# Autodesk Inventor assembly: Assembly
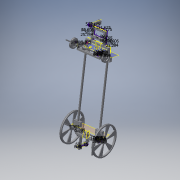
[picture p0: Inventor's stored thumbnail of the model, 180x180]
Saved by Autodesk Inventor 2018 (Build 220112000, 112)
## iProperties
Created: 2017-11-06
Part Number: Assembly
Document SubType Name: Assembly
Designer: David Cutting
Author: David Cutting
## Documents named in this file (19)
- C:\Users\Prakash\Documents\Inventor\MousetrapGit\Assembly.iam
- C:\Users\Prakash\Documents\Inventor\MousetrapGit\frontChassis_final.ipt
- C:\Users\Prakash\Documents\Inventor\MousetrapGit\carbonFiberTube.ipt
- C:\Users\Prakash\Documents\Inventor\MousetrapGit\clampCap.ipt
- C:\Users\Prakash\Documents\Inventor\MousetrapGit\rearChassis_final.ipt
- C:\Users\Prakash\Documents\Inventor\MousetrapGit\535018\bearings.ipt
- C:\Users\Prakash\Documents\Inventor\MousetrapGit\98873A200_MOISTURE-RESISTANT ACETAL THREADED ROD.ipt
- C:\Users\Prakash\Documents\Inventor\MousetrapGit\nutSecurer.ipt
- C:\Users\Prakash\Documents\Inventor\MousetrapGit\99223A029_ACETAL HEX NUT.ipt
- C:\Users\Prakash\Documents\Inventor\MousetrapGit\wheel.ipt
- C:\Users\Prakash\Documents\Inventor\MousetrapGit\spindleRod.ipt
- C:\Users\Prakash\Documents\Inventor\MousetrapGit\wheelSpindle.ipt
- C:\Users\Prakash\Documents\Inventor\MousetrapGit\intermediateSpindle.ipt
- C:\Users\Prakash\Documents\Inventor\MousetrapGit\wingnut_final.ipt
- C:\Users\Prakash\Documents\Inventor\MousetrapGit\washeript.ipt
- C:\Users\Prakash\Documents\Inventor\MousetrapGit\smallWheel.ipt
- C:\Users\Prakash\Documents\Inventor\MousetrapGit\springPusherAssembly.iam
- C:\Users\Prakash\Documents\Inventor\MousetrapGit\rearSight.ipt
- C:\Users\Prakash\Documents\Inventor\MousetrapGit\frontSight.ipt
## Components (48 placed, 18 different names)
1. frontChassis_final:1 — Mate:1, Mate:2, Mate:3, Mate:4, Angle:3, Flush:3, Angle:4, Flush:4, Mate:16, Mate:17, Mate:18, Mate:19, Angle:8, Mate:113, Flush:11, Flush:12
2. carbonFiberTube:1 — Mate:1, Mate:2, Mate:6, Mate:9, Mate:10
3. carbonFiberTube:2 — Mate:3, Mate:4, Mate:5, Mate:7, Mate:8, Mate:11
4. clampCap:1 — Mate:8, Angle:1, Flush:1
5. clampCap:2 — Mate:9, Angle:2, Flush:2
6. rearChassis_final:1 — Mate:5, Mate:6, Mate:7, Angle:1, Flush:1, Angle:2, Flush:2, Mate:96, Mate:97, Mate:99, Mate:109, Angle:9, Mate:114, Flush:13, Flush:14
7. clampCap:3 — Mate:10, Angle:3, Flush:3
8. clampCap:4 — Mate:11, Angle:4, Flush:4
9. bearings:1 — Mate:16, Mate:17, Mate:29, Mate:35
10. bearings:3 — Mate:18, Mate:19, Mate:28, Mate:39
11. bearings:4 — Mate:33, Mate:98, Mate:99
12. bearings:6 — Mate:30, Mate:37, Mate:97
13. 98873A200_MOISTURE-RESISTANT ACETAL THREADED ROD:1 — Mate:30, Mate:32, Mate:36, Mate:40, Mate:42, Mate:64, Mate:65, Mate:76, Mate:79, Mate:80, Mate:82, Mate:93, Mate:95, Mate:96, Flush:10, Mate:98, Mate:108, Mate:110
14. 98873A200_MOISTURE-RESISTANT ACETAL THREADED ROD:2 — Mate:28, Mate:29, Mate:34, Mate:38, Mate:44, Mate:46, Mate:63, Mate:66, Mate:67, Mate:77, Mate:81, Mate:83, Mate:84, Flush:8, Mate:102, Mate:104, Mate:111, Mate:112
15. nutSecurer:1 — Mate:34, Mate:35, Mate:47
16. nutSecurer:2 — Mate:36, Mate:37, Mate:41
17. nutSecurer:3 — Mate:32, Mate:33, Mate:43
18. nutSecurer:4 — Mate:38, Mate:39, Mate:45
19. 99223A029_ACETAL HEX NUT:1 — Mate:40, Mate:41, Mate:68
20. 99223A029_ACETAL HEX NUT:2 — Mate:42, Mate:43, Mate:69
21. 99223A029_ACETAL HEX NUT:3 — Mate:46, Mate:47, Mate:70
22. 99223A029_ACETAL HEX NUT:4 — Mate:44, Mate:45, Mate:71
23. wheel:2 — Mate:104, Mate:105, Mate:106
24. wheel:4 — Mate:102, Mate:103, Mate:107
25. spindleRod:1 — Mate:54
26. intermediateSpindle:1 — Mate:54
27. wingnut_final:2 — Mate:58, Mate:59, Mate:60, Mate:61, Mate:63, Angle:8
28. 99223A029_ACETAL HEX NUT:6 — Mate:58, Mate:59, Mate:60, Mate:61
29. 99223A029_ACETAL HEX NUT:7 — Mate:64, Mate:68, Mate:94
30. 99223A029_ACETAL HEX NUT:8 — Mate:65, Mate:69, Mate:101
31. 99223A029_ACETAL HEX NUT:9 — Mate:67, Mate:71, Mate:107
32. 99223A029_ACETAL HEX NUT:10 — Mate:66, Mate:70, Mate:106
33. 99223A029_ACETAL HEX NUT:11 — Mate:77, Mate:91, Flush:8
34. 99223A029_ACETAL HEX NUT:12 — Mate:76, Mate:89, Flush:10
35. 99223A029_ACETAL HEX NUT:13 — Mate:79, Mate:90
36. washeript:1 — Mate:82, Mate:90, Mate:100
37. washeript:2 — Mate:81, Mate:91, Mate:103
38. washeript:4 — Mate:80, Mate:89
39. washeript:5 — Mate:83, Mate:92, Mate:105
40. 99223A029_ACETAL HEX NUT:14 — Mate:84, Mate:92
41. smallWheel:1 — Mate:95, Mate:100, Mate:101
42. smallWheel:2 — Mate:93, Mate:94
43. springPusherAssembly:3 [sub-assembly] — Mate:108, Mate:109
44. wingnut_final:3 — Mate:110, Angle:9
45. springPusherAssembly:4 [sub-assembly] — Mate:111
46. wheelSpindle:1 — Mate:112
47. rearSight:1 — Mate:113, Flush:11, Flush:12
48. frontSight:1 — Mate:114, Flush:13, Flush:14
## Relationships (98: Mate 82, Flush 10, Angle 6)
- Mate:1: frontChassis_final:1 ↔ carbonFiberTube:1
- Mate:2: frontChassis_final:1 ↔ carbonFiberTube:1
- Mate:3: frontChassis_final:1 ↔ carbonFiberTube:2
- Mate:4: frontChassis_final:1 ↔ carbonFiberTube:2
- Mate:5: carbonFiberTube:2 ↔ rearChassis_final:1
- Mate:6: carbonFiberTube:1 ↔ rearChassis_final:1
- Mate:7: carbonFiberTube:2 ↔ rearChassis_final:1
- Mate:8: carbonFiberTube:2 ↔ clampCap:1
- Angle:1 (0 deg): clampCap:1 ↔ rearChassis_final:1
- Flush:1: clampCap:1 ↔ rearChassis_final:1
- Mate:9: carbonFiberTube:1 ↔ clampCap:2
- Angle:2 (0 deg): clampCap:2 ↔ rearChassis_final:1
- Flush:2: clampCap:2 ↔ rearChassis_final:1
- Mate:10: carbonFiberTube:1 ↔ clampCap:3
- Angle:3 (0 deg): frontChassis_final:1 ↔ clampCap:3
- Flush:3: frontChassis_final:1 ↔ clampCap:3
- Mate:11: carbonFiberTube:2 ↔ clampCap:4
- Angle:4 (0 deg): frontChassis_final:1 ↔ clampCap:4
- Flush:4: frontChassis_final:1 ↔ clampCap:4
- Mate:16: frontChassis_final:1 ↔ bearings:1
- Mate:17: frontChassis_final:1 ↔ bearings:1
- Mate:18: frontChassis_final:1 ↔ bearings:3
- Mate:19: frontChassis_final:1 ↔ bearings:3
- Mate:28: bearings:3 ↔ 98873A200_MOISTURE-RESISTANT ACETAL THREADED ROD:2
- Mate:29: bearings:1 ↔ 98873A200_MOISTURE-RESISTANT ACETAL THREADED ROD:2
- Mate:30: bearings:6 ↔ 98873A200_MOISTURE-RESISTANT ACETAL THREADED ROD:1
- Mate:32: 98873A200_MOISTURE-RESISTANT ACETAL THREADED ROD:1 ↔ nutSecurer:3
- Mate:33: bearings:4 ↔ nutSecurer:3
- Mate:34: 98873A200_MOISTURE-RESISTANT ACETAL THREADED ROD:2 ↔ nutSecurer:1
- Mate:35: bearings:1 ↔ nutSecurer:1
- Mate:36: 98873A200_MOISTURE-RESISTANT ACETAL THREADED ROD:1 ↔ nutSecurer:2
- Mate:37: bearings:6 ↔ nutSecurer:2
- Mate:38: 98873A200_MOISTURE-RESISTANT ACETAL THREADED ROD:2 ↔ nutSecurer:4
- Mate:39: bearings:3 ↔ nutSecurer:4
- Mate:40: 98873A200_MOISTURE-RESISTANT ACETAL THREADED ROD:1 ↔ 99223A029_ACETAL HEX NUT:1
- Mate:41: nutSecurer:2 ↔ 99223A029_ACETAL HEX NUT:1
- Mate:42: 98873A200_MOISTURE-RESISTANT ACETAL THREADED ROD:1 ↔ 99223A029_ACETAL HEX NUT:2
- Mate:43: nutSecurer:3 ↔ 99223A029_ACETAL HEX NUT:2
- Mate:44: 98873A200_MOISTURE-RESISTANT ACETAL THREADED ROD:2 ↔ 99223A029_ACETAL HEX NUT:4
- Mate:45: nutSecurer:4 ↔ 99223A029_ACETAL HEX NUT:4
- Mate:46: 98873A200_MOISTURE-RESISTANT ACETAL THREADED ROD:2 ↔ 99223A029_ACETAL HEX NUT:3
- Mate:47: nutSecurer:1 ↔ 99223A029_ACETAL HEX NUT:3
- Mate:54: spindleRod:1 ↔ intermediateSpindle:1
- Mate:58: wingnut_final:2 ↔ 99223A029_ACETAL HEX NUT:6
- Mate:59: wingnut_final:2 ↔ 99223A029_ACETAL HEX NUT:6
- Mate:60: wingnut_final:2 ↔ 99223A029_ACETAL HEX NUT:6
- Mate:61: wingnut_final:2 ↔ 99223A029_ACETAL HEX NUT:6
- Mate:63: 98873A200_MOISTURE-RESISTANT ACETAL THREADED ROD:2 ↔ wingnut_final:2
- Angle:8 (0 deg): frontChassis_final:1 ↔ wingnut_final:2
- Mate:64: 98873A200_MOISTURE-RESISTANT ACETAL THREADED ROD:1 ↔ 99223A029_ACETAL HEX NUT:7
- Mate:65: 98873A200_MOISTURE-RESISTANT ACETAL THREADED ROD:1 ↔ 99223A029_ACETAL HEX NUT:8
- Mate:66: 98873A200_MOISTURE-RESISTANT ACETAL THREADED ROD:2 ↔ 99223A029_ACETAL HEX NUT:10
- Mate:67: 98873A200_MOISTURE-RESISTANT ACETAL THREADED ROD:2 ↔ 99223A029_ACETAL HEX NUT:9
- Mate:68: 99223A029_ACETAL HEX NUT:1 ↔ 99223A029_ACETAL HEX NUT:7
- Mate:69: 99223A029_ACETAL HEX NUT:2 ↔ 99223A029_ACETAL HEX NUT:8
- Mate:70: 99223A029_ACETAL HEX NUT:3 ↔ 99223A029_ACETAL HEX NUT:10
- Mate:71: 99223A029_ACETAL HEX NUT:4 ↔ 99223A029_ACETAL HEX NUT:9
- Mate:76: 98873A200_MOISTURE-RESISTANT ACETAL THREADED ROD:1 ↔ 99223A029_ACETAL HEX NUT:12
- Mate:77: 98873A200_MOISTURE-RESISTANT ACETAL THREADED ROD:2 ↔ 99223A029_ACETAL HEX NUT:11
- Mate:79: 98873A200_MOISTURE-RESISTANT ACETAL THREADED ROD:1 ↔ 99223A029_ACETAL HEX NUT:13
- Mate:80: 98873A200_MOISTURE-RESISTANT ACETAL THREADED ROD:1 ↔ washeript:4
- Mate:81: 98873A200_MOISTURE-RESISTANT ACETAL THREADED ROD:2 ↔ washeript:2
- Mate:82: 98873A200_MOISTURE-RESISTANT ACETAL THREADED ROD:1 ↔ washeript:1
- Mate:83: 98873A200_MOISTURE-RESISTANT ACETAL THREADED ROD:2 ↔ washeript:5
- Mate:84: 98873A200_MOISTURE-RESISTANT ACETAL THREADED ROD:2 ↔ 99223A029_ACETAL HEX NUT:14
- Mate:89: 99223A029_ACETAL HEX NUT:12 ↔ washeript:4
- Mate:90: 99223A029_ACETAL HEX NUT:13 ↔ washeript:1
- Mate:91: 99223A029_ACETAL HEX NUT:11 ↔ washeript:2
- Mate:92: washeript:5 ↔ 99223A029_ACETAL HEX NUT:14
- Flush:8: 98873A200_MOISTURE-RESISTANT ACETAL THREADED ROD:2 ↔ 99223A029_ACETAL HEX NUT:11
- Mate:93: 98873A200_MOISTURE-RESISTANT ACETAL THREADED ROD:1 ↔ smallWheel:2
- Mate:94: 99223A029_ACETAL HEX NUT:7 ↔ smallWheel:2
- Mate:95: 98873A200_MOISTURE-RESISTANT ACETAL THREADED ROD:1 ↔ smallWheel:1
- Mate:96: rearChassis_final:1 ↔ 98873A200_MOISTURE-RESISTANT ACETAL THREADED ROD:1
- Mate:97: rearChassis_final:1 ↔ bearings:6
- Flush:10: 98873A200_MOISTURE-RESISTANT ACETAL THREADED ROD:1 ↔ 99223A029_ACETAL HEX NUT:12
- Mate:98: bearings:4 ↔ 98873A200_MOISTURE-RESISTANT ACETAL THREADED ROD:1
- Mate:99: rearChassis_final:1 ↔ bearings:4
- Mate:100: washeript:1 ↔ smallWheel:1
- Mate:101: 99223A029_ACETAL HEX NUT:8 ↔ smallWheel:1
- Mate:102: 98873A200_MOISTURE-RESISTANT ACETAL THREADED ROD:2 ↔ wheel:4
- Mate:103: wheel:4 ↔ washeript:2
- Mate:104: 98873A200_MOISTURE-RESISTANT ACETAL THREADED ROD:2 ↔ wheel:2
- Mate:105: wheel:2 ↔ washeript:5
- Mate:106: wheel:2 ↔ 99223A029_ACETAL HEX NUT:10
- Mate:107: wheel:4 ↔ 99223A029_ACETAL HEX NUT:9
- Mate:108: 98873A200_MOISTURE-RESISTANT ACETAL THREADED ROD:1 ↔ springPusherAssembly:3
- Mate:109: rearChassis_final:1 ↔ springPusherAssembly:3
- Mate:110: 98873A200_MOISTURE-RESISTANT ACETAL THREADED ROD:1 ↔ wingnut_final:3
- Angle:9 (0 deg): rearChassis_final:1 ↔ wingnut_final:3
- Mate:111: 98873A200_MOISTURE-RESISTANT ACETAL THREADED ROD:2 ↔ springPusherAssembly:4
- Mate:112: 98873A200_MOISTURE-RESISTANT ACETAL THREADED ROD:2 ↔ wheelSpindle:1
- Mate:113: frontChassis_final:1 ↔ rearSight:1
- Flush:11: frontChassis_final:1 ↔ rearSight:1
- Flush:12: frontChassis_final:1 ↔ rearSight:1
- Mate:114: rearChassis_final:1 ↔ frontSight:1
- Flush:13: rearChassis_final:1 ↔ frontSight:1
- Flush:14: rearChassis_final:1 ↔ frontSight:1
